# Autodesk Inventor assembly: RSX deck corrected
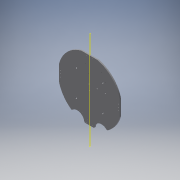
[picture p0: Inventor's stored thumbnail of the model, 180x180]
Saved by Autodesk Inventor 2017 (Build 210142000, 142)
## iProperties
Created: 2017-05-04
Part Number: RSX deck corrected
Document SubType Name: Assembly
Designer: qupec
Author: qupec
## Documents named in this file (2)
- D:\UMD Near Space\star\CAD\Mechanical\RSX deck corrected.iam
- D:\UMD Near Space\star\CAD\Mechanical\CapTech\CADD\CADD\RSX Assembly\RSX Deck.ipt
## Components (1 placed, 1 different names)
1. RSX Deck:1 — Mate:1, Flush:1
## Relationships (3: Mate 2, Flush 1)
- Mate:1: RSX Deck:1
- Flush:1 (-165.5877 mm): RSX Deck:1
- Mate:2
